# Autodesk Inventor assembly: Sestava
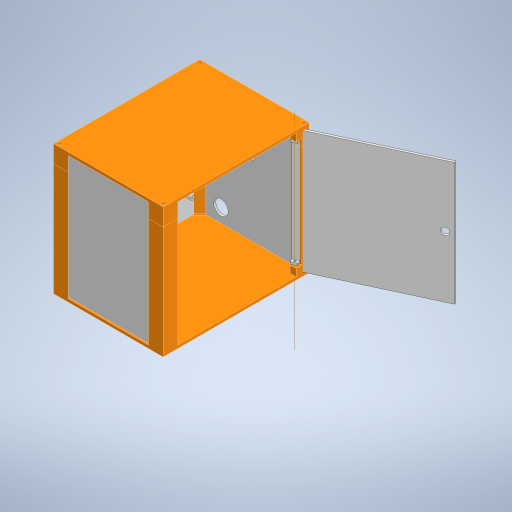
[picture p0: Inventor's stored thumbnail of the model, 512x512]
Saved by Autodesk Inventor 2024.3 (Build 283343000, 343)
## iProperties
Created: 2025-03-25
Part Number: Sestava
Document SubType Name: Assembly
Designer: admin
Author: admin
## Documents named in this file (7)
- D:\[05] Zaloha\[05] Stredni\[01] Prace a Materialy\[06] KYB\Rocnikovka\Rozvadec\Sestava.iam
- D:\[05] Zaloha\[05] Stredni\[01] Prace a Materialy\[06] KYB\Rocnikovka\Rozvadec\Cabinet - bottom.ipt
- D:\[05] Zaloha\[05] Stredni\[01] Prace a Materialy\[06] KYB\Rocnikovka\Rozvadec\Cabinet - top.ipt
- D:\[05] Zaloha\[05] Stredni\[01] Prace a Materialy\[06] KYB\Rocnikovka\Rozvadec\Cabinet - back.ipt
- D:\[05] Zaloha\[05] Stredni\[01] Prace a Materialy\[06] KYB\Rocnikovka\Rozvadec\Cabinet - left.ipt
- D:\[05] Zaloha\[05] Stredni\[01] Prace a Materialy\[06] KYB\Rocnikovka\Rozvadec\Cabinet - right.ipt
- D:\[05] Zaloha\[05] Stredni\[01] Prace a Materialy\[06] KYB\Rocnikovka\Rozvadec\Cabinet - door.ipt
## Components (6 placed, 6 different names)
1. Cabinet - bottom:1 — Proti sobě:1, Proti sobě:2, Proti sobě:3, Proti sobě:4, Proti sobě:5, Proti sobě:6, Souměrnost:1, Souměrnost:2, Souměrnost:3, Souměrnost:4, Souměrnost:5, Souměrnost:6, Souměrnost:7, Souměrnost:8, Souměrnost:9, Proti sobě:16, Souměrnost:10, Proti sobě:19
2. Cabinet - top:1 — Proti sobě:4, Proti sobě:5, Proti sobě:6, Souměrnost:1, Souměrnost:2, Souměrnost:3, Souměrnost:4, Souměrnost:6, Souměrnost:8, Souměrnost:9, Souměrnost:10
3. Cabinet - back:1 — Proti sobě:7, Proti sobě:8, Proti sobě:9, Souměrnost:5, Souměrnost:7
4. Cabinet - left:1 — Proti sobě:10, Proti sobě:11, Proti sobě:12
5. Cabinet - right:1 — Proti sobě:13, Proti sobě:14, Proti sobě:15
6. Cabinet - door:1 — Proti sobě:17, Proti sobě:18, Proti sobě:19
## Relationships (29: Mate 19, Symmetry 10)
- Proti sobě:1 [Mate]: Cabinet - bottom:1
- Proti sobě:2 [Mate]: Cabinet - bottom:1
- Proti sobě:3 [Mate]: Cabinet - bottom:1
- Proti sobě:4 [Mate]: Cabinet - bottom:1 ↔ Cabinet - top:1
- Proti sobě:5 [Mate]: Cabinet - bottom:1 ↔ Cabinet - top:1
- Proti sobě:6 [Mate]: Cabinet - bottom:1 ↔ Cabinet - top:1
- Souměrnost:1 [Symmetry]: Cabinet - bottom:1 ↔ Cabinet - top:1
- Proti sobě:7 [Mate]: Cabinet - back:1
- Souměrnost:2 [Symmetry]: Cabinet - bottom:1 ↔ Cabinet - top:1
- Proti sobě:8 [Mate]: Cabinet - back:1
- Souměrnost:3 [Symmetry]: Cabinet - bottom:1 ↔ Cabinet - top:1
- Proti sobě:9 [Mate]: Cabinet - back:1
- Souměrnost:4 [Symmetry]: Cabinet - bottom:1 ↔ Cabinet - top:1
- Proti sobě:10 [Mate]: Cabinet - left:1
- Souměrnost:5 [Symmetry]: Cabinet - bottom:1 ↔ Cabinet - back:1
- Proti sobě:11 [Mate]: Cabinet - left:1
- Souměrnost:6 [Symmetry]: Cabinet - bottom:1 ↔ Cabinet - top:1
- Proti sobě:12 [Mate]: Cabinet - left:1
- Souměrnost:7 [Symmetry]: Cabinet - bottom:1 ↔ Cabinet - back:1
- Proti sobě:13 [Mate]: Cabinet - right:1
- Souměrnost:8 [Symmetry]: Cabinet - bottom:1 ↔ Cabinet - top:1
- Proti sobě:14 [Mate]: Cabinet - right:1
- Souměrnost:9 [Symmetry]: Cabinet - bottom:1 ↔ Cabinet - top:1
- Proti sobě:15 [Mate]: Cabinet - right:1
- Proti sobě:16 [Mate]: Cabinet - bottom:1
- Proti sobě:17 [Mate]: Cabinet - door:1
- Souměrnost:10 [Symmetry]: Cabinet - bottom:1 ↔ Cabinet - top:1
- Proti sobě:18 [Mate]: Cabinet - door:1
- Proti sobě:19 [Mate]: Cabinet - bottom:1 ↔ Cabinet - door:1
